# Autodesk Inventor assembly: assembly
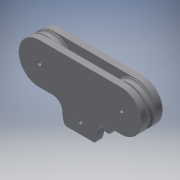
[picture p0: Inventor's stored thumbnail of the model, 180x180]
Saved by Autodesk Inventor 2016 (Build 200138000, 138)
## iProperties
Created: 2019-02-22
Part Number: assembly
Document SubType Name: Assembly
Designer: reesem783
Author: reesem783
## Documents named in this file (4)
- H:\Github\Zipline\Inventor\assembly.iam
- H:\Github\Zipline\Inventor\wheel.ipt
- H:\Github\Zipline\Inventor\casing.ipt
- H:\Github\Zipline\Inventor\bearing.ipt
## Components (8 placed, 3 different names)
1. casing:1 — Insert:1, Mate:1, Mate:2, Mate:10
2. casing:2 — Mate:9, Mate:10
3. bearing:1 — Mate:11
4. bearing:2 — Insert:1, Mate:12, Mate:14
5. bearing:3 — Mate:9, Mate:12
6. bearing:4 — Mate:1, Mate:2, Mate:11, Mate:13
7. wheel:1 — Mate:14
8. wheel:2 — Mate:13
## Relationships (9: Mate 8, Insert 1)
- Insert:1: casing:1 ↔ bearing:2
- Mate:1: casing:1 ↔ bearing:4
- Mate:2: casing:1 ↔ bearing:4
- Mate:9: casing:2 ↔ bearing:3
- Mate:10: casing:1 ↔ casing:2
- Mate:11: bearing:1 ↔ bearing:4
- Mate:12: bearing:2 ↔ bearing:3
- Mate:13: bearing:4 ↔ wheel:2
- Mate:14: bearing:2 ↔ wheel:1
